# Autodesk Inventor assembly: Intake
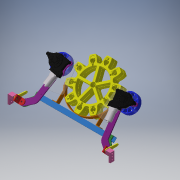
[picture p0: Inventor's stored thumbnail of the model, 180x180]
Saved by Autodesk Inventor 2017 (Build 210142000, 142)
## iProperties
Created: 2017-01-12
Part Number: Intake
Document SubType Name: Assembly
Designer: Ben
Author: Ben
## Documents named in this file (14)
- C:\Users\Ben\Desktop\Projects\2017 Robot\Gear Intake\Intake.iam
- C:\Users\Ben\Desktop\Projects\2017 Robot\Gear Intake\Intake Arms.ipt
- C:\Users\Ben\Desktop\Projects\2017 Robot\Gear Intake\Gear solid.iam
- C:\Users\Ben\Desktop\Projects\2017 Robot\Gear Intake\Corner Hinge.ipt
- C:\Users\Ben\Desktop\Projects\2017 Robot\Gear Intake\Gear Plates.ipt
- C:\Users\Ben\Desktop\Projects\2017 Robot\Gear Intake\Cross Arms.ipt
- C:\Users\Ben\Desktop\Projects\2017 Robot\Gear Intake\Cross Brace.ipt
- C:\Users\Ben\Desktop\Projects\2017 Robot\Gear Intake\Half moon catch.ipt
- C:\Users\Ben\Desktop\Projects\2017 Robot\Gear Intake\SW3dPS-Denso Window Motor Left.ipt
- C:\Users\Ben\Desktop\Projects\2017 Robot\Gear Intake\User Library-Denso Window Motor Right.ipt
- C:\Users\Ben\Desktop\Projects\2017 Robot\Gear Intake\torque arm.ipt
- C:\Users\Ben\Desktop\Projects\2017 Robot\Gear Intake\am-3480+4IN+Compliant+Wheel.iam
- C:\Users\Ben\Desktop\Projects\2017 Robot\Gear Intake\.375 bushing.ipt
- C:\Users\Ben\Desktop\Projects\2017 Robot\Gear Intake\Hinge Block 2.ipt
## Components (21 placed, 13 different names)
1. Intake Arms:1 — Insert:5, Mate:13, Symmetry:1, Flush:4, Insert:12, Mate:19, Angle:1, Insert:16
2. Intake Arms:2 — Insert:9, Mate:14, Symmetry:1, Flush:5, Insert:13, Mate:21, Mate:22, Angle:2, Insert:17
3. Gear solid:1 [sub-assembly] — Mate:9, Mate:18
4. Corner Hinge:1 — Insert:5, Flush:1, Mate:15, Insert:14, Mate:23
5. Corner Hinge:2 — Insert:9, Flush:1, Mate:15, Insert:15, Mate:24
6. Gear Plates:1 — Mate:13, Flush:4
7. Gear Plates:2 — Mate:14, Flush:5
8. Cross Arms:1 — Insert:12, Flush:6
9. Cross Arms:2 — Insert:13, Flush:6, Mate:16, Flush:7, Flush:8
10. Cross Brace:1 — Mate:16, Flush:7, Flush:8, Mate:17, Flush:9
11. Half moon catch:1 — Mate:17, Flush:9, Flush:10, Mate:18
12. SW3dPS-Denso Window Motor Left:1 — Mate:19, Angle:1
13. User Library-Denso Window Motor Right:1 — Mate:21, Mate:22, Angle:2
14. torque arm:1 — Insert:14, Mate:23, Insert:18
15. torque arm:2 — Insert:15, Insert:19, Mate:24
16. am-3480+4IN+Compliant+Wheel:1 [sub-assembly] — Insert:16
17. am-3480+4IN+Compliant+Wheel:2 [sub-assembly] — Insert:17
18. .375 bushing:1 — Insert:18, Insert:20
19. .375 bushing:2 — Insert:19, Insert:21
20. Hinge Block 2:1 — Insert:20, Flush:11, Mate:25, Symmetry:2, Mate:26
21. Hinge Block 2:2 — Insert:21, Flush:11, Symmetry:2
## Relationships (39: Mate 14, Insert 12, Flush 9, Symmetry 2, Angle 2)
- Mate:9: Gear solid:1
- Insert:5 (6.35 mm): Intake Arms:1 ↔ Corner Hinge:1
- Insert:9 (6.35 mm): Intake Arms:2 ↔ Corner Hinge:2
- Flush:1: Corner Hinge:1 ↔ Corner Hinge:2
- Mate:13: Intake Arms:1 ↔ Gear Plates:1
- Mate:14: Intake Arms:2 ↔ Gear Plates:2
- Symmetry:1: Intake Arms:1 ↔ Intake Arms:2
- Flush:4 (6.35 mm): Intake Arms:1 ↔ Gear Plates:1
- Flush:5 (6.35 mm): Intake Arms:2 ↔ Gear Plates:2
- Mate:15 (-539.75 mm): Corner Hinge:1 ↔ Corner Hinge:2
- Insert:12 (3.175 mm): Intake Arms:1 ↔ Cross Arms:1
- Insert:13 (3.175 mm): Intake Arms:2 ↔ Cross Arms:2
- Flush:6: Cross Arms:1 ↔ Cross Arms:2
- Mate:16: Cross Arms:2 ↔ Cross Brace:1
- Flush:7: Cross Arms:2 ↔ Cross Brace:1
- Flush:8: Cross Arms:2 ↔ Cross Brace:1
- Mate:17: Cross Brace:1 ↔ Half moon catch:1
- Flush:9: Cross Brace:1 ↔ Half moon catch:1
- Flush:10: Half moon catch:1
- Mate:18: Gear solid:1 ↔ Half moon catch:1
- Mate:19: Intake Arms:1 ↔ SW3dPS-Denso Window Motor Left:1
- Angle:1 (0 deg): Intake Arms:1 ↔ SW3dPS-Denso Window Motor Left:1
- Mate:21: Intake Arms:2 ↔ User Library-Denso Window Motor Right:1
- Mate:22: Intake Arms:2 ↔ User Library-Denso Window Motor Right:1
- Angle:2 (0 deg): Intake Arms:2 ↔ User Library-Denso Window Motor Right:1
- Insert:14: Corner Hinge:1 ↔ torque arm:1
- Insert:15: Corner Hinge:2 ↔ torque arm:2
- Insert:16 (7.62 mm): Intake Arms:1 ↔ am-3480+4IN+Compliant+Wheel:1
- Insert:17 (7.62 mm): Intake Arms:2 ↔ am-3480+4IN+Compliant+Wheel:2
- Mate:23: Corner Hinge:1 ↔ torque arm:1
- Insert:18: torque arm:1 ↔ .375 bushing:1
- Insert:19: torque arm:2 ↔ .375 bushing:2
- Insert:20 (1.5875 mm): .375 bushing:1 ↔ Hinge Block 2:1
- Insert:21 (1.5875 mm): .375 bushing:2 ↔ Hinge Block 2:2
- Flush:11: Hinge Block 2:1 ↔ Hinge Block 2:2
- Mate:24: Corner Hinge:2 ↔ torque arm:2
- Mate:25 (57.658 mm): Hinge Block 2:1
- Symmetry:2: Hinge Block 2:1 ↔ Hinge Block 2:2
- Mate:26 (60.325 mm): Hinge Block 2:1
